# Autodesk Inventor assembly: untitled.brd
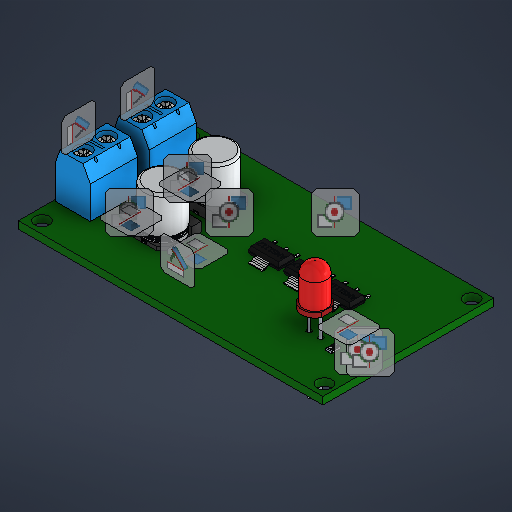
[picture p0: Inventor's stored thumbnail of the model, 512x512]
Saved by Autodesk Inventor 2025 (Build 290162000, 162)
## iProperties
Created: 2023-03-06
Part Number: untitled.brd
Document SubType Name: Assembly
Designer: Иван Петров
Author: Иван Петров
## Documents named in this file (7)
- D:\Projects\OmniBot\design\000.009 - Бортовой источник питания 3V3 СБ.iam
- D:\Projects\OmniBot\design\standart_components\Capacitors smd\05_NICHICON_8X10_NEWARK_58R3566_ENSAMBLE.ipt
- D:\Projects\OmniBot\design\standart_components\Terminal Block 2P.ipt
- D:\Projects\OmniBot\design\standart_components\LED-Red.ipt
- D:\Projects\OmniBot\design\standart_components\smd resistors\0R.iam
- D:\Projects\OmniBot\design\standart_components\AMS1117.ipt
- D:\Projects\OmniBot\design\000.009.001 - Плата печатная.ipt
## Components (10 placed, 10 different names)
1. 000.008.001 - Плата печатная
2. C9_2 — Совмещение:16, Угол:4, Заподлицо:1
3. C10_3 — Совмещение:16, Угол:4, Заподлицо:1
4. J1_5
5. J2_7
6. LED2_9
7. R6_11 [sub-assembly]
8. U1_13
9. U2_15
10. U3_17
## Relationships (16: Mate 11, Angle 4, Flush 1)
- [Angle] (0 deg): 000.008.001 - Плата печатная ↔ J1_5
- [Angle] (0 deg): 000.008.001 - Плата печатная ↔ J2_7
- [Mate]: 000.008.001 - Плата печатная ↔ J1_5
- [Mate]: 000.008.001 - Плата печатная ↔ J1_5
- [Mate]: 000.008.001 - Плата печатная ↔ J2_7
- [Mate]: 000.008.001 - Плата печатная ↔ J2_7
- [Mate]: 000.008.001 - Плата печатная ↔ LED2_9
- [Mate]: 000.008.001 - Плата печатная ↔ LED2_9
- [Mate] (5 mm): 000.008.001 - Плата печатная ↔ LED2_9
- [Mate]: 000.008.001 - Плата печатная ↔ C10_3
- [Mate] (-13.461 mm): 000.008.001 - Плата печатная ↔ C10_3
- [Mate] (-17.729 mm): 000.008.001 - Плата печатная ↔ C10_3
- Совмещение:16 [Mate] (11.179 mm): C9_2 ↔ C10_3
- [Angle] (0 deg): 000.008.001 - Плата печатная ↔ C10_3
- Угол:4 [Angle] (0 deg): C9_2 ↔ C10_3
- Заподлицо:1 [Flush]: C9_2 ↔ C10_3
